# Autodesk Inventor assembly: 3S Battery Assembly
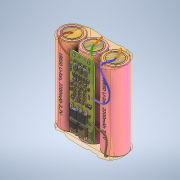
[picture p0: Inventor's stored thumbnail of the model, 180x180]
Saved by Autodesk Inventor 2022.1 (Build 261234020, 234B)
## iProperties
Created: 2021-07-28
Part Number: 3S Battery Assembly
Document SubType Name: Assembly
Designer: LJ
Mass: 180 g
Surface Area: 269.459 cm^2
Volume: 122.521 cm^3
Author: LJ
## Documents named in this file (5)
- C:\Users\LJ\Fusion\Optikal Secondary Payload\CubeSat 2021\Workspace\Battery\3S Battery Assembly.iam
- C:\Users\LJ\Fusion\Optikal Secondary Payload\CubeSat 2021\Workspace\Battery\3S BMS.ipt
- C:\Users\LJ\Fusion\Optikal Secondary Payload\CubeSat 2021\Workspace\Battery\18650.ipt
- C:\Users\LJ\Fusion\Optikal Secondary Payload\CubeSat 2021\Workspace\Battery\3S Battery Assembly\AIP\Cable and Harness\3S Battery Assembly.Harness1.iam
- C:\Users\LJ\Fusion\Optikal Secondary Payload\CubeSat 2021\Workspace\Battery\Kapton.ipt
## Components (6 placed, 4 different names)
1. 3S BMS:1 — Angle:1, Angle:2, Flush:5, Tangent:3, Flush:6
2. 18650:1 — Tangent:1, Flush:1, Flush:3, Flush:7
3. 18650:2 — Tangent:1, Tangent:2, Flush:1, Flush:2, Flush:3, Flush:4, Angle:1, Angle:2, Flush:5, Tangent:3, Flush:6
4. 18650:3 — Tangent:2, Flush:2, Flush:4, Flush:8
5. Harness1 [sub-assembly]
6. Kapton:1 — Flush:7, Flush:8
## Relationships (13: Flush 8, Tangent 3, Angle 2)
- Tangent:1: 18650:1 ↔ 18650:2
- Tangent:2: 18650:2 ↔ 18650:3
- Flush:1: 18650:1 ↔ 18650:2
- Flush:2: 18650:2 ↔ 18650:3
- Flush:3: 18650:1 ↔ 18650:2
- Flush:4: 18650:2 ↔ 18650:3
- Angle:1 (0 deg): 3S BMS:1 ↔ 18650:2
- Angle:2 (180 deg): 3S BMS:1 ↔ 18650:2
- Flush:5: 3S BMS:1 ↔ 18650:2
- Tangent:3: 3S BMS:1 ↔ 18650:2
- Flush:6 (2.5 mm): 3S BMS:1 ↔ 18650:2
- Flush:7: 18650:1 ↔ Kapton:1
- Flush:8: 18650:3 ↔ Kapton:1
